# Autodesk Inventor assembly: step mother_MIR
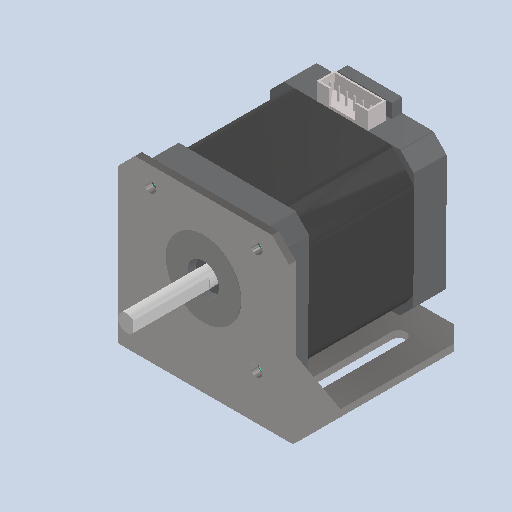
[picture p0: Inventor's stored thumbnail of the model, 512x512]
Saved by Autodesk Inventor 2025.1 (Build 291241000, 241)
## iProperties
Created: 2024-11-05
Part Number: step mother_MIR
Document SubType Name: Assembly
Designer: pedro
Author: pedro
## Documents named in this file (3)
- C:\Users\pedro\Documents\1-CoisasSerias\UTFPR\2024-2\Oficina\Estrutura\step mother_MIR.iam
- C:\Users\pedro\Documents\1-CoisasSerias\UTFPR\2024-2\Oficina\Estrutura\Pecas Prontas\temp\nema17-mounting-l-bracket-1.snapshot.2\NEMA17MountingLBracket_MIR.ipt
- C:\Users\pedro\Documents\1-CoisasSerias\UTFPR\2024-2\Oficina\Estrutura\Pecas Prontas\setp motor\nema-17-stepper-motor-17hs8401-1.snapshot.7\NEMA17 17HS8401\NEMA17 17HS8401\NEMA17 17HS8401_MIR.ipt
## Components (2 placed, 2 different names)
1. NEMA17MountingLBracket_MIR:1 — Coincidente:2, Coincidente:1
2. NEMA17 17HS8401_MIR:1 — Coincidente:2, Coincidente:1
## Relationships (2: Mate 2)
- Coincidente:2 [Mate]: NEMA17MountingLBracket_MIR:1 ↔ NEMA17 17HS8401_MIR:1
- Coincidente:1 [Mate]: NEMA17MountingLBracket_MIR:1 ↔ NEMA17 17HS8401_MIR:1
